# Autodesk Inventor assembly: __VK_Stopper
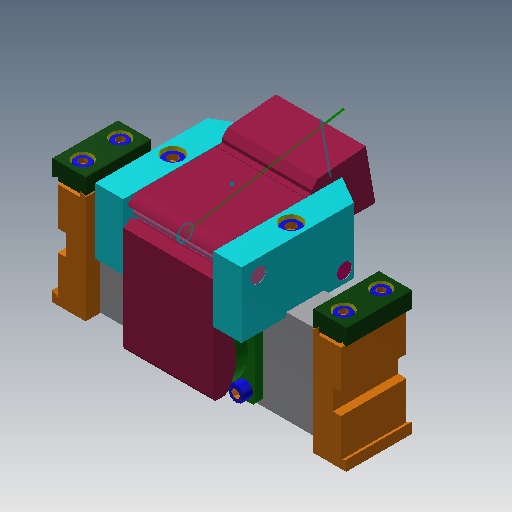
[picture p0: Inventor's stored thumbnail of the model, 512x512]
Saved by Autodesk Inventor 2019 (Build 230136000, 136)
## iProperties
Created: 2023-11-18
Part Number: __VK_Stopper
Material: Generisch
Document SubType Name: Assembly
Designer: RP
Author: RP
## Documents named in this file (3)
- C:\Users\RP\Documents\Inventor\Projekt_Angelspule\_Verkettung\__VK_Stopper.iam
- C:\Users\RP\Documents\Inventor\Projekt_Angelspule\_Verkettung\__VK_Stopper_Basis.ipt
- C:\Users\RP\Documents\Inventor\Projekt_Angelspule\_Verkettung\__VK_Stopper_Klinke.ipt
## Components (2 placed, 2 different names)
1. __VK_Stopper_Basis:1 — Fluchtend:2, Mitte_Werkstückträger, Fluchtend:4, Passend:1, Tangential:1, Tangential:2, Fluchtend:5
2. __VK_Stopper_Klinke:1 — Fluchtend:4, Passend:1, Tangential:1, Tangential:2
## Relationships (7: Flush 4, Tangent 2, Mate 1)
- Fluchtend:2 [Flush]: __VK_Stopper_Basis:1
- Mitte_Werkstückträger [Flush] (142.7424 mm): __VK_Stopper_Basis:1
- Fluchtend:4 [Flush]: __VK_Stopper_Basis:1 ↔ __VK_Stopper_Klinke:1
- Passend:1 [Mate]: __VK_Stopper_Basis:1 ↔ __VK_Stopper_Klinke:1
- Tangential:1: __VK_Stopper_Basis:1 ↔ __VK_Stopper_Klinke:1
- Tangential:2: __VK_Stopper_Basis:1 ↔ __VK_Stopper_Klinke:1
- Fluchtend:5 [Flush] (2.2196 mm): __VK_Stopper_Basis:1
